# Autodesk Inventor assembly: RightFootUnit
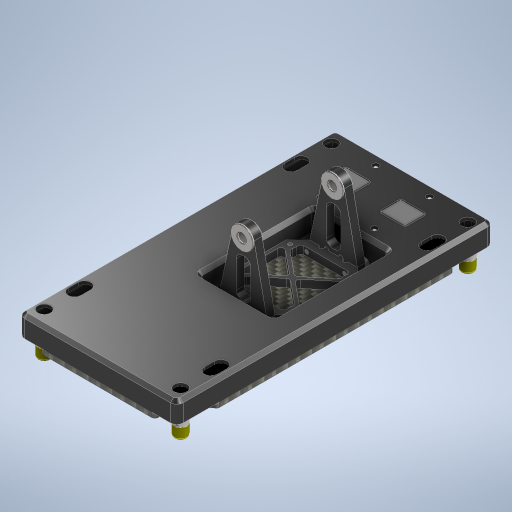
[picture p0: Inventor's stored thumbnail of the model, 512x512]
Saved by Autodesk Inventor 2024.2 (Build 282272000, 272)
## iProperties
Created: 2024-01-07
Part Number: RightFootUnit
Document SubType Name: Assembly
Designer: Masato Kubotera
Mass: 224.174 g
Surface Area: 1225.51 cm^2
Volume: 154.973 cm^3
Density: 1.44653 g/cm^3
Author: Masato Kubotera
## Documents named in this file (15)
- C:\Users\masato\OneDrive - Chiba Institute of Technology\CIT Brains\RoboCup2024\Mechanic\SUSTAINA-OP2-DEV1\NativeFiles\Boby\LowerLimb\Feet\RightFootUnit.iam
- C:\Users\masato\OneDrive - Chiba Institute of Technology\CIT Brains\RoboCup2024\Mechanic\SUSTAINA-OP2-DEV1\NativeFiles\Boby\LowerLimb\LegRollSliderFrame.ipt
- C:\Users\masato\OneDrive - Chiba Institute of Technology\CIT Brains\RoboCup2024\Mechanic\SUSTAINA-OP2-DEV1\NativeFiles\Boby\COTS\Bushes\GFM-0608-06.ipt
- C:\Users\masato\OneDrive - Chiba Institute of Technology\CIT Brains\RoboCup2024\Mechanic\SUSTAINA-OP2-DEV1\NativeFiles\Boby\COTS\Washers\Metal\UUW-0614-05H.ipt
- C:\Users\masato\OneDrive - Chiba Institute of Technology\CIT Brains\RoboCup2024\Mechanic\SUSTAINA-OP2-DEV1\NativeFiles\Boby\COTS\Screws\CapScrew\UC-0310.ipt
- C:\Users\masato\OneDrive - Chiba Institute of Technology\CIT Brains\RoboCup2024\Mechanic\SUSTAINA-OP2-DEV1\NativeFiles\Boby\LowerLimb\Feet\FootBraceFrame.ipt
- C:\Users\masato\OneDrive - Chiba Institute of Technology\CIT Brains\RoboCup2024\Mechanic\SUSTAINA-OP2-DEV1\NativeFiles\Boby\COTS\Screws\CapScrew\UC-0308.ipt
- C:\Users\masato\OneDrive - Chiba Institute of Technology\CIT Brains\RoboCup2024\Mechanic\SUSTAINA-OP2-DEV1\NativeFiles\Boby\COTS\MisumiComponents\URLM8\URLM8.iam
- C:\Users\masato\OneDrive - Chiba Institute of Technology\CIT Brains\RoboCup2024\Mechanic\SUSTAINA-OP2-DEV1\NativeFiles\Boby\COTS\ElectronicComponents\SC700-40kg.ipt
- C:\Users\masato\OneDrive - Chiba Institute of Technology\CIT Brains\RoboCup2024\Mechanic\SUSTAINA-OP2-DEV1\NativeFiles\Boby\LowerLimb\Feet\RightFootCover.ipt
- C:\Users\masato\OneDrive - Chiba Institute of Technology\CIT Brains\RoboCup2024\Mechanic\SUSTAINA-OP2-DEV1\NativeFiles\Boby\COTS\Washers\Resin\TT-0614-05.ipt
- C:\Users\masato\OneDrive - Chiba Institute of Technology\CIT Brains\RoboCup2024\Mechanic\SUSTAINA-OP2-DEV1\NativeFiles\Boby\CustomPCBs\SUSTAINA-STRAINGAUGE-SENSING-BOARD.ipt
- C:\Users\masato\OneDrive - Chiba Institute of Technology\CIT Brains\RoboCup2024\Mechanic\SUSTAINA-OP2-DEV1\NativeFiles\Boby\LowerLimb\Feet\FootSoleFrame_MIR.ipt
- C:\Users\masato\OneDrive - Chiba Institute of Technology\CIT Brains\RoboCup2024\Mechanic\SUSTAINA-OP2-DEV1\NativeFiles\Boby\COTS\Nuts\UNT-03.ipt
- C:\Users\masato\OneDrive - Chiba Institute of Technology\CIT Brains\RoboCup2024\Mechanic\SUSTAINA-OP2-DEV1\NativeFiles\Boby\COTS\Spacers\WBN-305.ipt
## Components (52 placed, 14 different names)
1. UNT-03:1 — Insert:52
2. UNT-03:2 — Insert:51
3. UNT-03:3 — Insert:48
4. UNT-03:4 — Insert:47
5. UNT-03:5 — Insert:50
6. UNT-03:6 — Insert:49
7. UNT-03:7 — Insert:46
8. UNT-03:8 — Insert:45
9. UNT-03:9 — Insert:54
10. UNT-03:10 — Insert:53
11. UNT-03:11 — Insert:56
12. UNT-03:12 — Insert:55
13. WBN-305:1 — Insert:59, Insert:62
14. WBN-305:2 — Insert:58
15. WBN-305:3 — Insert:60
16. WBN-305:4 — Insert:57, Insert:61
17. LegRollSliderFrame:1 — Mate:1, Angle:1, Flush:2, Flush:3, Insert:1, Insert:3, Insert:7, Insert:8, Insert:11, Insert:12, Mate:2
18. LegRollSliderFrame:2 — Flush:2, Flush:3, Insert:2, Insert:4, Insert:9, Insert:10, Insert:13, Insert:14
19. FootBraceFrame:1 — Insert:11, Insert:12, Insert:13, Insert:14, Insert:15, Insert:16, Insert:17, Insert:18
20. FootSoleFrame_MIR:1 — Insert:15, Insert:16, Insert:17, Insert:18, Insert:19, Insert:20, Insert:21, Insert:22, Insert:23, Insert:24, Insert:25, Insert:26, Insert:27, Insert:28, Insert:29, Insert:30, Flush:8, Flush:7, Flush:5, Insert:45, Insert:46, Insert:47, Insert:48, Insert:49, Insert:50, Insert:51, Insert:52, Insert:53, Insert:54, Insert:55, Insert:56, Insert:57, Insert:58, Insert:59, Insert:60
21. SUSTAINA-STRAINGAUGE-SENSING-BOARD:1 — Insert:61, Insert:62
22. RightFootCover:1 — Flush:8, Flush:7, Flush:5
23. GFM-0608-06:1 — Insert:1
24. GFM-0608-06:2 — Insert:2
25. SC700-40kg:1 — Insert:23, Insert:24, Insert:31, Insert:42, Insert:38
26. SC700-40kg:2 — Insert:25, Insert:26, Insert:32, Insert:41, Insert:37
27. SC700-40kg:3 — Insert:27, Insert:28, Insert:33, Insert:40, Insert:44
28. SC700-40kg:4 — Insert:29, Insert:30, Insert:34, Insert:43, Insert:39
29. UC-0308:5 — Insert:41
30. UC-0308:9 — Insert:37
31. UC-0308:6 — Insert:42
32. UC-0308:10 — Insert:38
33. UC-0308:7 — Insert:43
34. UC-0308:12 — Insert:39
35. UC-0308:8 — Insert:44
36. UC-0308:11 — Insert:40
37. UC-0310:1 — Insert:7
38. UC-0310:2 — Insert:8
39. UC-0310:3 — Insert:9
40. UC-0310:4 — Insert:10
41. UC-0308:1 — Insert:19
42. UC-0308:2 — Insert:20
43. UC-0308:3 — Insert:21
44. UC-0308:4 — Insert:22
45. URLM8:1 [sub-assembly] — Insert:31
46. URLM8:2 [sub-assembly] — Insert:32
47. URLM8:3 [sub-assembly] — Insert:33
48. URLM8:4 [sub-assembly] — Insert:34
49. TT-0614-05:1 — Insert:3, Insert:5
50. TT-0614-05:2 — Insert:4, Insert:6
51. UUW-0614-05H:1 — Insert:5
52. UUW-0614-05H:2 — Insert:6
## Relationships (68: Insert 60, Flush 5, Mate 2, Angle 1)
- Mate:1: LegRollSliderFrame:1
- Angle:1 (180 deg): LegRollSliderFrame:1
- Flush:2: LegRollSliderFrame:1 ↔ LegRollSliderFrame:2
- Flush:3: LegRollSliderFrame:1 ↔ LegRollSliderFrame:2
- Insert:1: LegRollSliderFrame:1 ↔ GFM-0608-06:1
- Insert:2: LegRollSliderFrame:2 ↔ GFM-0608-06:2
- Insert:3: LegRollSliderFrame:1 ↔ TT-0614-05:1
- Insert:4: LegRollSliderFrame:2 ↔ TT-0614-05:2
- Insert:5: TT-0614-05:1 ↔ UUW-0614-05H:1
- Insert:6: TT-0614-05:2 ↔ UUW-0614-05H:2
- Insert:7: LegRollSliderFrame:1 ↔ UC-0310:1
- Insert:8: LegRollSliderFrame:1 ↔ UC-0310:2
- Insert:9: LegRollSliderFrame:2 ↔ UC-0310:3
- Insert:10: LegRollSliderFrame:2 ↔ UC-0310:4
- Insert:11: LegRollSliderFrame:1 ↔ FootBraceFrame:1
- Insert:12: LegRollSliderFrame:1 ↔ FootBraceFrame:1
- Insert:13: LegRollSliderFrame:2 ↔ FootBraceFrame:1
- Insert:14: LegRollSliderFrame:2 ↔ FootBraceFrame:1
- Mate:2 (16 mm): LegRollSliderFrame:1
- Insert:15: FootBraceFrame:1 ↔ FootSoleFrame_MIR:1
- Insert:16: FootBraceFrame:1 ↔ FootSoleFrame_MIR:1
- Insert:17: FootBraceFrame:1 ↔ FootSoleFrame_MIR:1
- Insert:18: FootBraceFrame:1 ↔ FootSoleFrame_MIR:1
- Insert:19: FootSoleFrame_MIR:1 ↔ UC-0308:1
- Insert:20: FootSoleFrame_MIR:1 ↔ UC-0308:2
- Insert:21: FootSoleFrame_MIR:1 ↔ UC-0308:3
- Insert:22: FootSoleFrame_MIR:1 ↔ UC-0308:4
- Insert:23: FootSoleFrame_MIR:1 ↔ SC700-40kg:1
- Insert:24: FootSoleFrame_MIR:1 ↔ SC700-40kg:1
- Insert:25: FootSoleFrame_MIR:1 ↔ SC700-40kg:2
- Insert:26: FootSoleFrame_MIR:1 ↔ SC700-40kg:2
- Insert:27: FootSoleFrame_MIR:1 ↔ SC700-40kg:3
- Insert:28: FootSoleFrame_MIR:1 ↔ SC700-40kg:3
- Insert:29: FootSoleFrame_MIR:1 ↔ SC700-40kg:4
- Insert:30: FootSoleFrame_MIR:1 ↔ SC700-40kg:4
- Insert:31: SC700-40kg:1 ↔ URLM8:1
- Insert:32: SC700-40kg:2 ↔ URLM8:2
- Insert:33: SC700-40kg:3 ↔ URLM8:3
- Insert:34: SC700-40kg:4 ↔ URLM8:4
- Insert:37: SC700-40kg:2 ↔ UC-0308:9
- Insert:38: SC700-40kg:1 ↔ UC-0308:10
- Insert:39: SC700-40kg:4 ↔ UC-0308:12
- Insert:40: SC700-40kg:3 ↔ UC-0308:11
- Insert:41: SC700-40kg:2 ↔ UC-0308:5
- Insert:42: SC700-40kg:1 ↔ UC-0308:6
- Insert:43: SC700-40kg:4 ↔ UC-0308:7
- Insert:44: SC700-40kg:3 ↔ UC-0308:8
- Flush:8: FootSoleFrame_MIR:1 ↔ RightFootCover:1
- Flush:7: FootSoleFrame_MIR:1 ↔ RightFootCover:1
- Flush:5: FootSoleFrame_MIR:1 ↔ RightFootCover:1
- Insert:45: UNT-03:8 ↔ FootSoleFrame_MIR:1
- Insert:46: UNT-03:7 ↔ FootSoleFrame_MIR:1
- Insert:47: UNT-03:4 ↔ FootSoleFrame_MIR:1
- Insert:48: UNT-03:3 ↔ FootSoleFrame_MIR:1
- Insert:49: UNT-03:6 ↔ FootSoleFrame_MIR:1
- Insert:50: UNT-03:5 ↔ FootSoleFrame_MIR:1
- Insert:51: UNT-03:2 ↔ FootSoleFrame_MIR:1
- Insert:52: UNT-03:1 ↔ FootSoleFrame_MIR:1
- Insert:53: UNT-03:10 ↔ FootSoleFrame_MIR:1
- Insert:54: UNT-03:9 ↔ FootSoleFrame_MIR:1
- Insert:55: UNT-03:12 ↔ FootSoleFrame_MIR:1
- Insert:56: UNT-03:11 ↔ FootSoleFrame_MIR:1
- Insert:57: WBN-305:4 ↔ FootSoleFrame_MIR:1
- Insert:58: WBN-305:2 ↔ FootSoleFrame_MIR:1
- Insert:59: WBN-305:1 ↔ FootSoleFrame_MIR:1
- Insert:60: WBN-305:3 ↔ FootSoleFrame_MIR:1
- Insert:61: WBN-305:4 ↔ SUSTAINA-STRAINGAUGE-SENSING-BOARD:1
- Insert:62: WBN-305:1 ↔ SUSTAINA-STRAINGAUGE-SENSING-BOARD:1
